# Autodesk Inventor assembly: PistonFrameMini
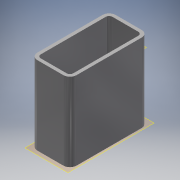
[picture p0: Inventor's stored thumbnail of the model, 180x180]
Saved by Autodesk Inventor 2016 (Build 200138000, 138)
## iProperties
Created: 2015-08-01
Part Number: PistonFrameMini
Document SubType Name: Assembly
Designer: myhome
Author: myhome
## Documents named in this file (2)
- C:\Users\myhome\Documents\Inventor\Printer\PistonFrame\PistonFeederFrameMini.iam
- C:\Users\myhome\Documents\Inventor\Printer\PistonFrame\DIN EN 10219-2 - 120 x 60 x 5  - 0.001.ipt
## Components (1 placed, 1 different names)
1. DIN EN 10219-2 - 120 x 60 x 5  - 0.001:1 — Flush:1
## Relationships (1: Flush 1)
- Flush:1: DIN EN 10219-2 - 120 x 60 x 5  - 0.001:1
